# Autodesk Inventor assembly: StereoCabinet
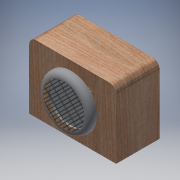
[picture p0: Inventor's stored thumbnail of the model, 180x180]
Saved by Autodesk Inventor 2017 (Build 210142000, 142)
## iProperties
Created: 2018-07-25
Part Number: StereoCabinet
Document SubType Name: Assembly
Designer: Jake
Author: Jake
## Documents named in this file (4)
- C:\Users\Jake\git\CAD-Projects\StereoCabinet\StereoCabinet.iam
- C:\Users\Jake\git\CAD-Projects\StereoCabinet\speakerBox.ipt
- C:\Users\Jake\git\CAD-Projects\StereoCabinet\speaker.ipt
- C:\Users\Jake\git\CAD-Projects\StereoCabinet\speakerGrill.ipt
## Components (3 placed, 3 different names)
1. speakerBox:1 — Rotational:1
2. speaker:1 — Rotational:1, Rotational:2
3. speakerGrill:1 — Rotational:2
## Relationships (2: RevoluteJoint 2)
- Rotational:1 [RevoluteJoint]: speakerBox:1 ↔ speaker:1
- Rotational:2 [RevoluteJoint]: speaker:1 ↔ speakerGrill:1
